# Autodesk Inventor assembly: gear_Assembly
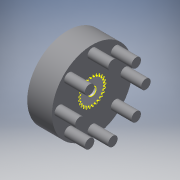
[picture p0: Inventor's stored thumbnail of the model, 180x180]
Saved by Autodesk Inventor 2018 (Build 220112000, 112)
## iProperties
Created: 2019-01-07
Part Number: gear_Assembly
Material: 一般
Document SubType Name: Assembly
Designer: lowyu
Author: lowyu
## Documents named in this file (3)
- C:\Users\lowyu\Desktop\HAND\シャッターハンド\卒論\originals\parts\gear_Assembly.iam
- C:\Users\lowyu\Desktop\HAND\シャッターハンド\卒論\originals\parts\moto_gear.ipt
- C:\Users\lowyu\Desktop\HAND\シャッターハンド\サーボモータ\gear.ipt
## Components (2 placed, 2 different names)
1. moto_gear:1 — メイト:1
2. gear:1 — メイト:1
## Relationships (1: Mate 1)
- メイト:1 [Mate]: moto_gear:1 ↔ gear:1
